# Autodesk Inventor assembly: fork_MIR
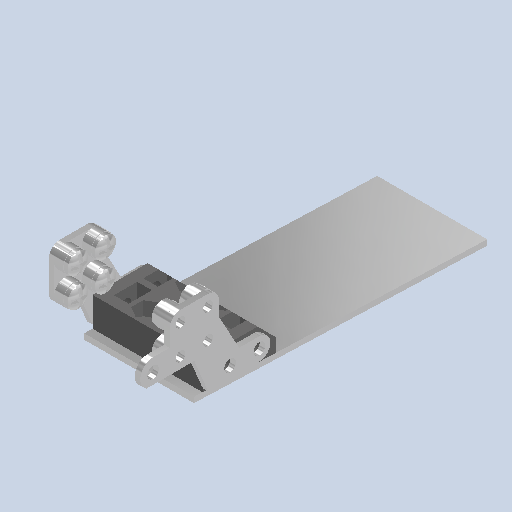
[picture p0: Inventor's stored thumbnail of the model, 512x512]
Saved by Autodesk Inventor 2024.1 (Build 281209000, 209)
## iProperties
Created: 2025-01-18
Part Number: fork_MIR
Document SubType Name: Assembly
Designer: hibik
Author: hibik
## Documents named in this file (6)
- C:\Users\hibik\Documents\Robomech\RESCUE\ORCA\hard\fork\right\fork_MIR.iam
- C:\Users\hibik\Documents\Robomech\RESCUE\ORCA\hard\fork\right\fork_middle_MIR.ipt
- C:\Users\hibik\Documents\Robomech\RESCUE\ORCA\hard\fork\right\fork_inside_MIR.ipt
- C:\Users\hibik\Documents\Robomech\RESCUE\ORCA\hard\fork\right\fork_outside_MIR.ipt
- C:\Users\hibik\Documents\Robomech\RESCUE\ORCA\hard\std_parts\bearing_3_6_2.5_MIR.ipt
- C:\Users\hibik\Documents\Robomech\RESCUE\ORCA\hard\fork\right\fork_fork_MIR.ipt
## Components (12 placed, 5 different names)
1. fork_middle_MIR:1 — 挿入:4, 挿入:3, 挿入:2, 挿入:1, 挿入:16, 挿入:15, 挿入:14, 挿入:13
2. fork_inside_MIR:1 — 挿入:4, 挿入:3, 挿入:9, 挿入:10, 挿入:12, 挿入:11
3. fork_outside_MIR:1 — 挿入:2, 挿入:1, 挿入:5, 挿入:6, 挿入:8, 挿入:7
4. bearing_3_6_2.5_MIR:1 — 挿入:5
5. bearing_3_6_2.5_MIR:2 — 挿入:6
6. bearing_3_6_2.5_MIR:3 — 挿入:8
7. bearing_3_6_2.5_MIR:4 — 挿入:7
8. bearing_3_6_2.5_MIR:5 — 挿入:9
9. bearing_3_6_2.5_MIR:6 — 挿入:10
10. bearing_3_6_2.5_MIR:7 — 挿入:12
11. bearing_3_6_2.5_MIR:8 — 挿入:11
12. fork_fork_MIR:1 — 挿入:16, 挿入:15, 挿入:14, 挿入:13
## Relationships (16: Insert 16)
- 挿入:4 [Insert]: fork_middle_MIR:1 ↔ fork_inside_MIR:1
- 挿入:3 [Insert]: fork_middle_MIR:1 ↔ fork_inside_MIR:1
- 挿入:2 [Insert]: fork_middle_MIR:1 ↔ fork_outside_MIR:1
- 挿入:1 [Insert]: fork_middle_MIR:1 ↔ fork_outside_MIR:1
- 挿入:5 [Insert]: fork_outside_MIR:1 ↔ bearing_3_6_2.5_MIR:1
- 挿入:6 [Insert]: fork_outside_MIR:1 ↔ bearing_3_6_2.5_MIR:2
- 挿入:8 [Insert]: fork_outside_MIR:1 ↔ bearing_3_6_2.5_MIR:3
- 挿入:7 [Insert]: fork_outside_MIR:1 ↔ bearing_3_6_2.5_MIR:4
- 挿入:9 [Insert]: fork_inside_MIR:1 ↔ bearing_3_6_2.5_MIR:5
- 挿入:10 [Insert]: fork_inside_MIR:1 ↔ bearing_3_6_2.5_MIR:6
- 挿入:12 [Insert]: fork_inside_MIR:1 ↔ bearing_3_6_2.5_MIR:7
- 挿入:11 [Insert]: fork_inside_MIR:1 ↔ bearing_3_6_2.5_MIR:8
- 挿入:16 [Insert]: fork_middle_MIR:1 ↔ fork_fork_MIR:1
- 挿入:15 [Insert]: fork_middle_MIR:1 ↔ fork_fork_MIR:1
- 挿入:14 [Insert]: fork_middle_MIR:1 ↔ fork_fork_MIR:1
- 挿入:13 [Insert]: fork_middle_MIR:1 ↔ fork_fork_MIR:1
